# Autodesk Inventor assembly: Hauptmodul
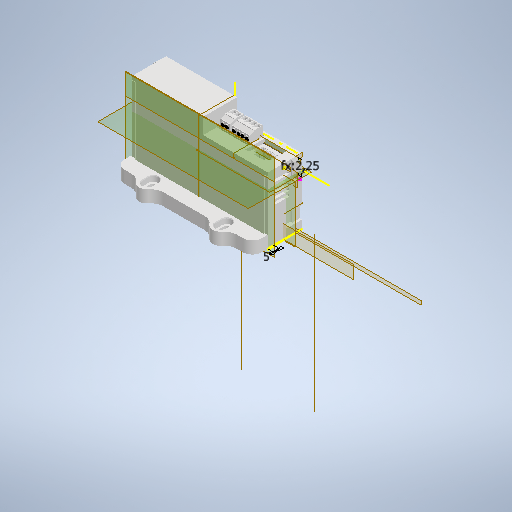
[picture p0: Inventor's stored thumbnail of the model, 512x512]
Saved by Autodesk Inventor 2025.2 (Build 292293000, 293)
## iProperties
Created: 2025-11-03
Part Number: Hauptmodul
Document SubType Name: Assembly
Designer: leowa
Author: leowa
## Documents named in this file (7)
- C:\Users\leowa\OneDrive - Fachhochschule Aachen\FH\8. Semester\CAN Tram CAD\Module\Hauptmodul.iam
- C:\Users\leowa\OneDrive - Fachhochschule Aachen\FH\8. Semester\CAN Tram CAD\Platinen\Hauptmodul\Hauptmodul\Hauptmodul.iam
- C:\Users\leowa\OneDrive - Fachhochschule Aachen\FH\8. Semester\CAN Tram CAD\Kaufteile\epp32-devkitc32u-wifi-ble-module-1.snapshot.1\ESP32-DevkitC32D\ESP32-DevkitC32D\ESP32-DevkitC32D.iam
- C:\Users\leowa\OneDrive - Fachhochschule Aachen\FH\8. Semester\CAN Tram CAD\Kaufteile\Terminalstecker 2fach\0395000002.iam
- C:\Users\leowa\OneDrive - Fachhochschule Aachen\FH\8. Semester\CAN Tram CAD\Kaufteile\Terminalstecker 4fach\0395000004.iam
- C:\Users\leowa\OneDrive - Fachhochschule Aachen\FH\8. Semester\CAN Tram CAD\Gehäuse\Hauptmodul Gehäuse V2.ipt
- C:\Users\leowa\OneDrive - Fachhochschule Aachen\FH\8. Semester\CAN Tram CAD\Gehäuse\Hauptmodul Deckel V2.ipt
## Components (6 placed, 6 different names)
1. Hauptmodul:1 [sub-assembly] — Passend:3, Fluchtend:1, Fluchtend:2, Passend:6, Passend:7, Passend:8, Passend:9, Passend:10, Passend:11, Passend:12, Passend:13, Passend:14
2. ESP32-DevkitC32D:1 [sub-assembly] — Passend:3, Fluchtend:1, Fluchtend:2
3. 0395000002:1 [sub-assembly] — Passend:7, Passend:9, Passend:11
4. 0395000004:1 [sub-assembly] — Passend:6, Passend:8, Passend:10
5. Hauptmodul Gehäuse V2:1 — Passend:12, Passend:13, Passend:14, Fluchtend:3, Fluchtend:4, Passend:15
6. Hauptmodul Deckel V2:1 — Fluchtend:3, Fluchtend:4, Passend:15
## Relationships (15: Mate 11, Flush 4)
- Passend:3 [Mate]: Hauptmodul:1 ↔ ESP32-DevkitC32D:1
- Fluchtend:1 [Flush]: Hauptmodul:1 ↔ ESP32-DevkitC32D:1
- Fluchtend:2 [Flush]: Hauptmodul:1 ↔ ESP32-DevkitC32D:1
- Passend:6 [Mate]: Hauptmodul:1 ↔ 0395000004:1
- Passend:7 [Mate]: Hauptmodul:1 ↔ 0395000002:1
- Passend:8 [Mate]: Hauptmodul:1 ↔ 0395000004:1
- Passend:9 [Mate]: Hauptmodul:1 ↔ 0395000002:1
- Passend:10 [Mate]: Hauptmodul:1 ↔ 0395000004:1
- Passend:11 [Mate]: Hauptmodul:1 ↔ 0395000002:1
- Passend:12 [Mate]: Hauptmodul:1 ↔ Hauptmodul Gehäuse V2:1
- Passend:13 [Mate]: Hauptmodul:1 ↔ Hauptmodul Gehäuse V2:1
- Passend:14 [Mate] (1 mm): Hauptmodul:1 ↔ Hauptmodul Gehäuse V2:1
- Fluchtend:3 [Flush]: Hauptmodul Gehäuse V2:1 ↔ Hauptmodul Deckel V2:1
- Fluchtend:4 [Flush]: Hauptmodul Gehäuse V2:1 ↔ Hauptmodul Deckel V2:1
- Passend:15 [Mate]: Hauptmodul Gehäuse V2:1 ↔ Hauptmodul Deckel V2:1
